# Autodesk Inventor assembly: Aircraft Preliminary Design and W+B
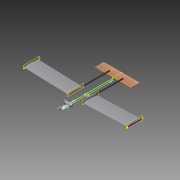
[picture p0: Inventor's stored thumbnail of the model, 180x180]
Saved by Autodesk Inventor 2015 (Build 190159000, 159)
## iProperties
Created: 2018-07-21
Part Number: Aircraft Preliminary Design and W+B
Document SubType Name: Assembly
Designer: Michael Gunderman
Author: Michael Gunderman
## Documents named in this file (8)
- C:\Users\Michael Gunderman\Documents\Special Projects\Echo 1\CAD work\Preliminary Shapes\Aircraft Preliminary Design and W+B.iam
- C:\Users\Michael Gunderman\Documents\Special Projects\Echo 1\CAD work\Systems\Electrical\Motor Turnigy G60 500kv.ipt
- C:\Users\Michael Gunderman\Documents\Special Projects\Echo 1\CAD work\Preliminary Shapes\Generic Wing 1.ipt
- C:\Users\Michael Gunderman\Documents\Special Projects\Echo 1\CAD work\Preliminary Shapes\Generic Tail 1.ipt
- C:\Users\Michael Gunderman\Documents\Special Projects\Echo 1\CAD work\Structures\500mm tube.ipt
- C:\Users\Michael Gunderman\Documents\Special Projects\Echo 1\CAD work\Preliminary Shapes\Generic Wing 1_MIR.ipt
- C:\Users\Michael Gunderman\Documents\Special Projects\Echo 1\CAD work\Structures\500mm tube_MIR.ipt
- C:\Users\Michael Gunderman\Documents\Special Projects\Echo 1\CAD work\Systems\Electrical\Flight Battery 5000 mah 5S.ipt
## Components (7 placed, 7 different names)
1. Motor Turnigy G60 500kv:1
2. Generic Wing 1:1 — Mate:1
3. Generic Tail 1:1 — Mate:2
4. 500mm tube:1
5. Generic Wing 1_MIR:1 — Mate:3
6. 500mm tube_MIR:1
7. Flight Battery 5000 mah 5S:1
## Relationships (4: Mate 3, Flush 1)
- Flush:1 (143 mm)
- Mate:1: Generic Wing 1:1
- Mate:2: Generic Tail 1:1
- Mate:3: Generic Wing 1_MIR:1
